# Autodesk Inventor assembly: 211-01
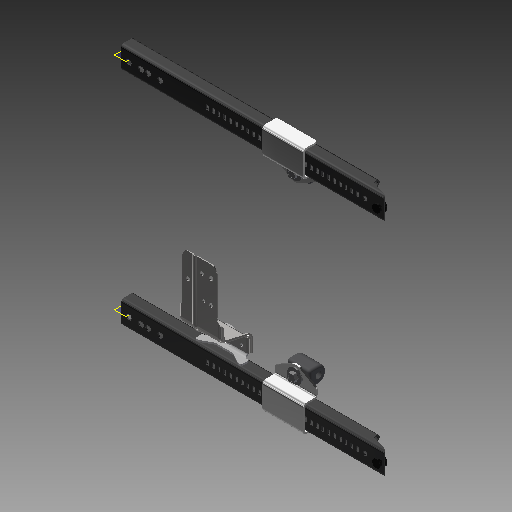
[picture p0: Inventor's stored thumbnail of the model, 512x512]
Saved by Autodesk Inventor 2019 (Build 230136000, 136)
## iProperties
Company: Autodesk Inc.
Created: 2007-12-24
Part Number: 211-01
Description: BOTTOM RAIL ASSEMBLY
Document SubType Name: Assembly
Designer: Autodesk Inc.
Mass: 2090.15 g
Surface Area: 2746.11 cm^2
Volume: 335.646 cm^3
Density: 6.22726 g/cm^3
Component Category: Lower Component
Author: Inventor
## Documents named in this file (8)
- C:\TEMP\Car Seat\Workspace\Bottom Rail Assembly_MIR.iam
- C:\TEMP\Car Seat\Workspace\Base Rail.ipt
- C:\TEMP\Car Seat\Workspace\Rail Slide.ipt
- C:\TEMP\Car Seat\Workspace\Ball Screw Mounting Block.ipt
- C:\TEMP\Car Seat\Workspace\Ball Screw Pin.ipt
- C:\TEMP\Car Seat\Workspace\Power Mounting Bracket_MIR.ipt
- C:\TEMP\Car Seat\Workspace\Floor Pin.ipt
- C:\TEMP\Car Seat\Workspace\Floor Mounting Bracket.ipt
## Components (12 placed, 7 different names)
1. Base Rail:1 — Flush:1, Mate:1, Flush:2, Flush:4, Mate:5, Mate:6, Angle:2, Angle:4, Mate:14, Mate:13, Mate:3
2. Base Rail:2 — Flush:2, Mate:2, Mate:7, Flush:3, Angle:1, Flush:6, Flush:5, Mate:9, Angle:3, Mate:12, Mate:15, Mate:4
3. Rail Slide:1 — Flush:4, Mate:5, Mate:6, Mate:8, Insert:1, Insert:4
4. Rail Slide:2 — Mate:7, Mate:8, Flush:3, Insert:2, Insert:3
5. Ball Screw Mounting Block:1 — Angle:1, Insert:2
6. Ball Screw Mounting Block:2 — Angle:2, Insert:1
7. Ball Screw Pin:1 — Insert:4
8. Ball Screw Pin:2 — Insert:3
9. Floor Mounting Bracket:1 — Flush:6, Flush:5, Mate:9, Mate:10, Insert:5
10. Power Mounting Bracket_MIR:1 — Mate:10, Insert:5
11. Floor Pin:1 — Angle:3, Mate:12, Mate:15
12. Floor Pin:2 — Angle:4, Mate:14, Mate:13
## Relationships (29: Mate 13, Flush 7, Insert 5, Angle 4)
- Flush:1 [Mate] (5.875 mm): Base Rail:1
- Mate:1: Base Rail:1
- Flush:2: Base Rail:1 ↔ Base Rail:2
- Mate:2: Base Rail:2
- Flush:4 (106 mm): Base Rail:1 ↔ Rail Slide:1
- Mate:5 (0.5 mm): Base Rail:1 ↔ Rail Slide:1
- Mate:6 [Flush]: Base Rail:1 ↔ Rail Slide:1
- Mate:7 (0.5 mm): Base Rail:2 ↔ Rail Slide:2
- Mate:8: Rail Slide:1 ↔ Rail Slide:2
- Flush:3 [Mate]: Base Rail:2 ↔ Rail Slide:2
- Angle:2 (90 deg): Base Rail:1 ↔ Ball Screw Mounting Block:2
- Insert:1: Rail Slide:1 ↔ Ball Screw Mounting Block:2
- Angle:1 (90 deg): Base Rail:2 ↔ Ball Screw Mounting Block:1
- Insert:2: Rail Slide:2 ↔ Ball Screw Mounting Block:1
- Insert:4: Rail Slide:1 ↔ Ball Screw Pin:1
- Insert:3: Rail Slide:2 ↔ Ball Screw Pin:2
- Flush:6 (-22 mm): Base Rail:2 ↔ Floor Mounting Bracket:1
- Flush:5 (125 mm): Base Rail:2 ↔ Floor Mounting Bracket:1
- Mate:9: Base Rail:2 ↔ Floor Mounting Bracket:1
- Mate:10: Floor Mounting Bracket:1 ↔ Power Mounting Bracket_MIR:1
- Insert:5: Floor Mounting Bracket:1 ↔ Power Mounting Bracket_MIR:1
- Angle:3 (0 deg): Base Rail:2 ↔ Floor Pin:1
- Mate:12: Base Rail:2 ↔ Floor Pin:1
- Mate:15: Base Rail:2 ↔ Floor Pin:1
- Angle:4 (0 deg): Base Rail:1 ↔ Floor Pin:2
- Mate:14: Base Rail:1 ↔ Floor Pin:2
- Mate:13: Base Rail:1 ↔ Floor Pin:2
- Mate:3 [Flush]: Base Rail:1
- Mate:4 [Flush]: Base Rail:2
